# Autodesk Inventor assembly: Wankel_Engine_V21-8
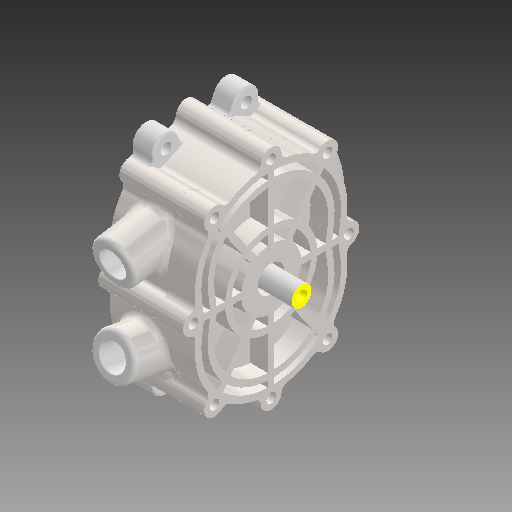
[picture p0: Inventor's stored thumbnail of the model, 512x512]
Saved by Autodesk Inventor 2020 (Build 240168000, 168)
## iProperties
Created: 2021-05-12
Part Number: Wankel_Engine_V21-8
Description: STEP AP214
Document SubType Name: Assembly
Designer: DDeGo
Sending System: SolidWorks 2020
Preprocessor: SwSTEP 2.0
Title: Wankel Engine V2(1-8).STEP
Revision Number: ANY
## Documents named in this file (7)
- C:\Users\DDeGo\Documents\Drew\Projects\AirWankelEngine\cad\IntegzaVersion\Wankel_Engine_Assy.iam
- C:\Users\DDeGo\Documents\Drew\Projects\AirWankelEngine\cad\IntegzaVersion\Body.ipt
- C:\Users\DDeGo\Documents\Drew\Projects\AirWankelEngine\cad\IntegzaVersion\Lid.ipt
- C:\Users\DDeGo\Documents\Drew\Projects\AirWankelEngine\cad\IntegzaVersion\Rotor.ipt
- C:\Users\DDeGo\Documents\Drew\Projects\AirWankelEngine\cad\hardware\6701 bearing.ipt
- C:\Users\DDeGo\Documents\Drew\Projects\AirWankelEngine\cad\hardware\MR85 bearing.ipt
- C:\Users\DDeGo\Documents\Drew\Projects\AirWankelEngine\cad\IntegzaVersion\Shaft.ipt
## Components (7 placed, 6 different names)
1. Body:1 — Mate:2, Mate:4, Mate:8, Mate:13, Mate:14, Mate:15
2. Lid:1 — Mate:12, Mate:13, Mate:14, Mate:15, Mate:16
3. Rotor:1 — Mate:6, Mate:8, Mate:9, Rotation:1
4. 6701 bearing:1 — Mate:5, Mate:6, Mate:9
5. MR85 bearing:1 — Mate:2, Mate:4, Mate:10, Mate:11
6. Shaft:1 — Mate:5, Mate:10, Mate:11, Rotation:1
7. MR85 bearing:2 — Mate:12, Mate:16
## Relationships (14: Mate 13, RelateRotation 1)
- Mate:2: Body:1 ↔ MR85 bearing:1
- Mate:4: Body:1 ↔ MR85 bearing:1
- Mate:5: 6701 bearing:1 ↔ Shaft:1
- Mate:6: Rotor:1 ↔ 6701 bearing:1
- Mate:8: Body:1 ↔ Rotor:1
- Mate:9: Rotor:1 ↔ 6701 bearing:1
- Mate:10: MR85 bearing:1 ↔ Shaft:1
- Mate:11: MR85 bearing:1 ↔ Shaft:1
- Mate:12: Lid:1 ↔ MR85 bearing:2
- Mate:13: Body:1 ↔ Lid:1
- Mate:14: Body:1 ↔ Lid:1
- Mate:15: Body:1 ↔ Lid:1
- Mate:16: Lid:1 ↔ MR85 bearing:2
- Rotation:1 [RelateRotation] (3 ul): Rotor:1 ↔ Shaft:1
